# Autodesk Inventor assembly: nc_nhk5
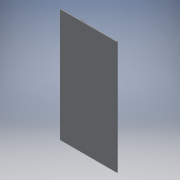
[picture p0: Inventor's stored thumbnail of the model, 180x180]
Saved by Autodesk Inventor 2019 (Build 230136000, 136)
## iProperties
Created: 2022-02-27
Part Number: nc_nhk5
Material: 一般
Document SubType Name: Assembly
Designer: yuta
Author: yuta
## Documents named in this file (4)
- C:\Users\yuta\Documents\NHK\nc_nhk5.iam
- C:\Users\yuta\Documents\NHK\NC.1.ipt
- C:\Users\yuta\Documents\NHK\nhk27.ipt
- C:\Users\yuta\Documents\NHK\nhk44.ipt
## Components (3 placed, 3 different names)
1. NC.1:1 — メイト:1, メイト:2
2. nhk27:1 — メイト:2
3. nhk44:1 — メイト:1
## Relationships (2: Mate 2)
- メイト:1 [Mate]: NC.1:1 ↔ nhk44:1
- メイト:2 [Mate]: NC.1:1 ↔ nhk27:1
